# Autodesk Inventor assembly: крыша
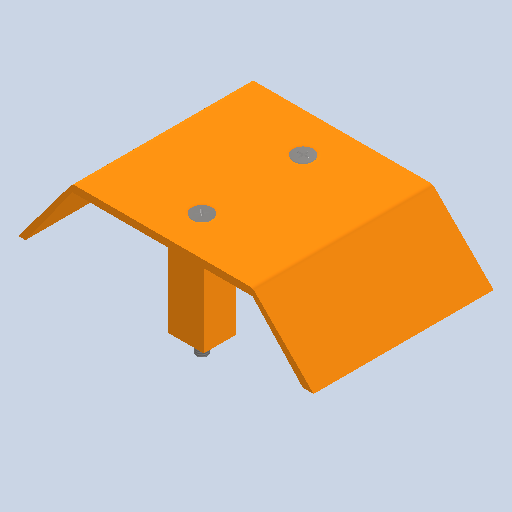
[picture p0: Inventor's stored thumbnail of the model, 512x512]
Saved by Autodesk Inventor 2022 (Build 260153000, 153)
## iProperties
Created: 2025-02-01
Part Number: крыша
Document SubType Name: Assembly
Designer: it
Author: it
## Documents named in this file (3)
- G:\машина\крыша.iam
- G:\машина\крыша1.ipt
- G:\abuyz lkz vfibyrb\Винт 2.M3-6gx30 ГОСТ 17475-80.ipt
## Components (3 placed, 2 different names)
1. крыша1:1 — Совмещение:3
2. Винт 2 ГОСТ 17475-80 M3 x 30:1 — Совмещение:3
3. Винт 2 ГОСТ 17475-80 M3 x 30:2
## Relationships (4: Mate 3, Flush 1)
- [Mate]: крыша1:1 ↔ Винт 2 ГОСТ 17475-80 M3 x 30:2
- [Mate]: крыша1:1 ↔ Винт 2 ГОСТ 17475-80 M3 x 30:2
- [Flush]: крыша1:1 ↔ Винт 2 ГОСТ 17475-80 M3 x 30:1
- Совмещение:3 [Mate]: крыша1:1 ↔ Винт 2 ГОСТ 17475-80 M3 x 30:1
